# Autodesk Inventor assembly: Left Internal Side Panel Assembly
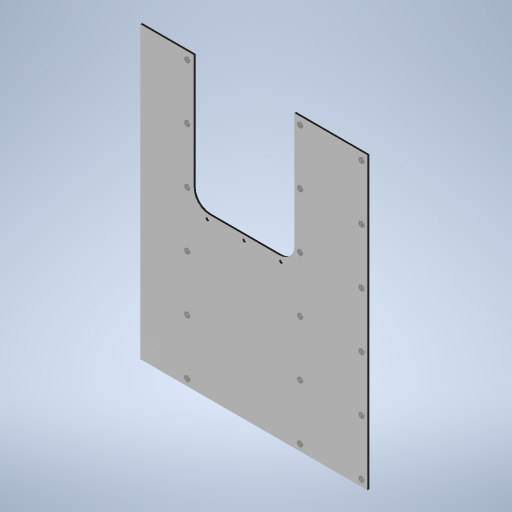
[picture p0: Inventor's stored thumbnail of the model, 512x512]
Saved by Autodesk Inventor 2024 (Build 280153000, 153)
## iProperties
Created: 2024-10-26
Part Number: Left Internal Side Panel Assembly
Document SubType Name: Assembly
Designer: Ishaan
Author: Ishaan
## Documents named in this file (4)
- E:\Projects\Axiom--IDEX-3D-Printer\CAD\08 - Side Panelling\Left Internal Side Panel Assembly.iam
- E:\Projects\Axiom--IDEX-3D-Printer\CAD\08 - Side Panelling\Side Internal Side Panel R2.ipt
- E:\Projects\Axiom--IDEX-3D-Printer\CAD\00 - COTS Components\Hardware\Low Profile M5x8.ipt
- E:\Projects\Axiom--IDEX-3D-Printer\CAD\00 - COTS Components\Hardware\M5 T SLOT NUT.ipt
## Components (37 placed, 3 different names)
1. Side Internal Side Panel R2:1 — Insert:1, Insert:2, Insert:3, Angle:1, Insert:4, Insert:5, Angle:2, Angle:3
2. Low Profile M5x8:13 — Insert:2
3. Low Profile M5x8:14
4. Low Profile M5x8:15
5. Low Profile M5x8:16
6. Low Profile M5x8:17
7. Low Profile M5x8:18
8. M5 T SLOT NUT:1 — Insert:3, Angle:1
9. M5 T SLOT NUT:3 — Insert:4, Angle:3
10. M5 T SLOT NUT:2 — Insert:5, Angle:2
11. M5 T SLOT NUT:4
12. M5 T SLOT NUT:5
13. M5 T SLOT NUT:6
14. M5 T SLOT NUT:7
15. M5 T SLOT NUT:8
16. M5 T SLOT NUT:9
17. M5 T SLOT NUT:10
18. M5 T SLOT NUT:11
19. M5 T SLOT NUT:12
20. M5 T SLOT NUT:13
21. M5 T SLOT NUT:14
22. M5 T SLOT NUT:15
23. M5 T SLOT NUT:16
24. M5 T SLOT NUT:17
25. M5 T SLOT NUT:18
26. Low Profile M5x8:1 — Insert:1
27. Low Profile M5x8:2
28. Low Profile M5x8:3
29. Low Profile M5x8:4
30. Low Profile M5x8:5
31. Low Profile M5x8:6
32. Low Profile M5x8:7
33. Low Profile M5x8:8
34. Low Profile M5x8:9
35. Low Profile M5x8:10
36. Low Profile M5x8:11
37. Low Profile M5x8:12
## Component patterns: (2 elements), (6 elements, first: Low Profile M5x8:13), (6 elements, first: M5 T SLOT NUT:1 + M5 T SLOT NUT:3 + M5 T SLOT NUT:2), (6 elements, first: Low Profile M5x8:1), Component Pattern 1:2 (6 elements)
## Relationships (8: Insert 5, Angle 3)
- Insert:1: Side Internal Side Panel R2:1 ↔ Low Profile M5x8:1
- Insert:2: Side Internal Side Panel R2:1 ↔ Low Profile M5x8:13
- Insert:3 (2 mm): Side Internal Side Panel R2:1 ↔ M5 T SLOT NUT:1
- Angle:1 (0 deg): Side Internal Side Panel R2:1 ↔ M5 T SLOT NUT:1
- Insert:4 (2 mm): Side Internal Side Panel R2:1 ↔ M5 T SLOT NUT:3
- Insert:5 (2 mm): Side Internal Side Panel R2:1 ↔ M5 T SLOT NUT:2
- Angle:2 (0 deg): Side Internal Side Panel R2:1 ↔ M5 T SLOT NUT:2
- Angle:3 (0 deg): Side Internal Side Panel R2:1 ↔ M5 T SLOT NUT:3
